# Autodesk Inventor assembly: sensorBoard
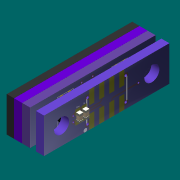
[picture p0: Inventor's stored thumbnail of the model, 180x180]
Saved by Autodesk Inventor 2016 SP1 (Build 200210100, 210)
## iProperties
Created: 2016-02-15
Part Number: sensorBoard
Document SubType Name: Assembly
Designer: sawai
Author: sawai
## Documents named in this file (6)
- C:\Users\sawai\OneDrive\projects\mppcSensorInterface\cad\sensorBoard.iam
- C:\Users\sawai\OneDrive\projects\mppcSensorInterface\cad\sensorBoardA\pcb.ipt
- C:\Users\sawai\OneDrive\projects\mppcSensorInterface\cad\sensorBoardB\boardB.iam
- C:\Users\sawai\OneDrive\projects\mppcSensorInterface\cad\sensorBoardC\boardC.iam
- C:\Users\sawai\OneDrive\projects\mppcSensorInterface\cad\sensorBoardA\groundGlassDisc.ipt
- C:\Users\sawai\OneDrive\projects\mppcSensorInterface\cad\sensorBoardA\lightGasket.ipt
## Components (5 placed, 5 different names)
1. pcb:1 — Flush:3, Flush:4, Mate:1, Flush:6, Flush:7, Mate:3, Mate:4
2. boardB:1 [sub-assembly] — Flush:1, Flush:2, Flush:3, Flush:4, Mate:2, Mate:3, Mate:5
3. boardC:1 [sub-assembly] — Flush:1, Flush:2, Mate:2
4. groundGlassDisc:1 — Mate:1, Mate:5
5. lightGasket:1 — Flush:6, Flush:7, Mate:4
## Relationships (11: Flush 6, Mate 5)
- Flush:1: boardB:1 ↔ boardC:1
- Flush:2: boardB:1 ↔ boardC:1
- Flush:3: pcb:1 ↔ boardB:1
- Flush:4: pcb:1 ↔ boardB:1
- Mate:1: pcb:1 ↔ groundGlassDisc:1
- Flush:6: pcb:1 ↔ lightGasket:1
- Flush:7: pcb:1 ↔ lightGasket:1
- Mate:2: boardB:1 ↔ boardC:1
- Mate:3: pcb:1 ↔ boardB:1
- Mate:4: pcb:1 ↔ lightGasket:1
- Mate:5: boardB:1 ↔ groundGlassDisc:1
